# Autodesk Inventor assembly: CARCASA_ESTRUCTURA_Y_CHAPAS
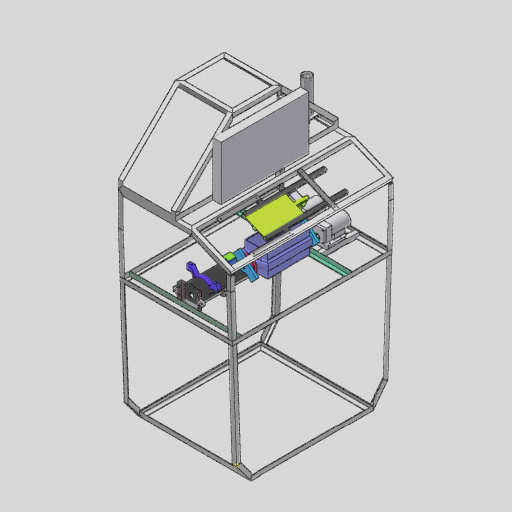
[picture p0: Inventor's stored thumbnail of the model, 512x512]
Saved by Autodesk Inventor 2024 (Build 280153000, 153)
## iProperties
Created: 2024-05-18
Part Number: CARCASA_ESTRUCTURA_Y_CHAPAS
Material: Generic
Document SubType Name: Assembly
Designer: Niler
Author: Niler
## Documents named in this file (7)
- C:\Users\Jhuliams\Documents\GitHub\RECICLADOR_MODELO_3D\VERSION_3_COMPLETA\CARCASA_ESTRUCTURA_Y_CHAPAS_1.iam
- C:\Users\Jhuliams\Documents\GitHub\RECICLADOR_MODELO_3D\VERSION_3_COMPLETA\ESTRUCTURA\ESTRUCTURA_COMPLETA.iam
- C:\Users\Jhuliams\Documents\GitHub\RECICLADOR_MODELO_3D\MECANISMO DE COMPACTADO\ENSAMBLE MECANISMO DE INGRESO.iam
- C:\Users\Jhuliams\Documents\GitHub\RECICLADOR_MODELO_3D\MECANISMO DE COMPACTADO\MECANISMO DE COMPACTADO.iam
- C:\Users\Jhuliams\Documents\GitHub\RECICLADOR_MODELO_3D\MECANISMO DE COMPACTADO\SEPARACION LATA-BOTELLA Y PAPEL.iam
- C:\Users\Jhuliams\Documents\GitHub\RECICLADOR_MODELO_3D\MECANISMO DE RECOMPENSA\RECOMPENSA.iam
- C:\Users\Jhuliams\Documents\GitHub\RECICLADOR_MODELO_3D\MECANISMO DE RECOMPENSA\PANTALLA.ipt
## Components (6 placed, 6 different names)
1. ESTRUCTURA_COMPLETA:1 [sub-assembly] — Mate:14, Mate:15, Mate:16, Mate:20, Mate:21, Mate:22, Mate:23, Flush:1, Flush:2, Mate:25, Flush:4, Mate:26
2. MECANISMO DE COMPACTADO:1 [sub-assembly] — Mate:14, Mate:15, Mate:16, Mate:24, Flush:3
3. RECOMPENSA:1 [sub-assembly] — Mate:20, Mate:21
4. PANTALLA:1 — Mate:22, Mate:23, Flush:1
5. ENSAMBLE MECANISMO DE INGRESO:1 [sub-assembly] — Flush:2, Mate:24, Mate:25
6. SEPARACION LATA-BOTELLA Y PAPEL:1 [sub-assembly] — Flush:3, Flush:4, Mate:26
## Relationships (14: Mate 10, Flush 4)
- Mate:14: ESTRUCTURA_COMPLETA:1 ↔ MECANISMO DE COMPACTADO:1
- Mate:15 (50 mm): ESTRUCTURA_COMPLETA:1 ↔ MECANISMO DE COMPACTADO:1
- Mate:16: ESTRUCTURA_COMPLETA:1 ↔ MECANISMO DE COMPACTADO:1
- Mate:20: ESTRUCTURA_COMPLETA:1 ↔ RECOMPENSA:1
- Mate:21 (100 mm): ESTRUCTURA_COMPLETA:1 ↔ RECOMPENSA:1
- Mate:22: ESTRUCTURA_COMPLETA:1 ↔ PANTALLA:1
- Mate:23: ESTRUCTURA_COMPLETA:1 ↔ PANTALLA:1
- Flush:1 (-120 mm): ESTRUCTURA_COMPLETA:1 ↔ PANTALLA:1
- Flush:2: ESTRUCTURA_COMPLETA:1 ↔ ENSAMBLE MECANISMO DE INGRESO:1
- Mate:24: MECANISMO DE COMPACTADO:1 ↔ ENSAMBLE MECANISMO DE INGRESO:1
- Mate:25: ESTRUCTURA_COMPLETA:1 ↔ ENSAMBLE MECANISMO DE INGRESO:1
- Flush:3 (-68.62 mm): MECANISMO DE COMPACTADO:1 ↔ SEPARACION LATA-BOTELLA Y PAPEL:1
- Flush:4 (-300 mm): ESTRUCTURA_COMPLETA:1 ↔ SEPARACION LATA-BOTELLA Y PAPEL:1
- Mate:26 (160 mm): ESTRUCTURA_COMPLETA:1 ↔ SEPARACION LATA-BOTELLA Y PAPEL:1
